# Autodesk Inventor assembly: 64mm_EDF
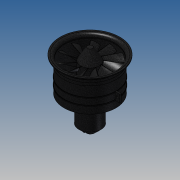
[picture p0: Inventor's stored thumbnail of the model, 180x180]
Saved by Autodesk Inventor 2015 (Build 190159000, 159)
## iProperties
Created: 2018-12-11
Part Number: 64mm_EDF
Document SubType Name: Assembly
Designer: USER
Author: USER
## Documents named in this file (5)
- D:\1102103229\碩士班\論文\Inventor\Drone_twincopterEDF_總組立\64mmEDF_總組立圖4.5\64mm_EDF_3D\64mm_EDF.iam
- D:\1102103229\碩士班\論文\Inventor\Drone_twincopterEDF_總組立\64mmEDF_總組立圖4.5\64mm_EDF_3D\64mm_motor.ipt
- D:\1102103229\碩士班\論文\Inventor\Drone_twincopterEDF_總組立\64mmEDF_總組立圖4.5\64mm_EDF_3D\64mm風扇本體.ipt
- D:\1102103229\碩士班\論文\Inventor\Drone_twincopterEDF_總組立\64mmEDF_總組立圖4.5\64mm_EDF_3D\64mm扇葉.ipt
- D:\1102103229\碩士班\論文\Inventor\Drone_twincopterEDF_總組立\64mmEDF_總組立圖4.5\64mm_EDF_3D\64mm導風口.ipt
## Components (4 placed, 4 different names)
1. 64mm_motor:1 — 貼合:2, 貼合:3, 旋轉:1
2. 64mm風扇本體:1 — 貼合:1, 貼合:2, 貼合:3, 貼合:4, 貼合:5, 齊平:1
3. 64mm扇葉:1 — 貼合:1, 齊平:1, 旋轉:1
4. 64mm導風口:1 — 貼合:4, 貼合:5
## Relationships (7: Mate 5, Flush 1, RelateRotation 1)
- 貼合:1 [Mate]: 64mm風扇本體:1 ↔ 64mm扇葉:1
- 貼合:2 [Mate]: 64mm_motor:1 ↔ 64mm風扇本體:1
- 貼合:3 [Mate]: 64mm_motor:1 ↔ 64mm風扇本體:1
- 貼合:4 [Mate]: 64mm風扇本體:1 ↔ 64mm導風口:1
- 貼合:5 [Mate]: 64mm風扇本體:1 ↔ 64mm導風口:1
- 齊平:1 [Flush] (-13 mm): 64mm風扇本體:1 ↔ 64mm扇葉:1
- 旋轉:1 [RelateRotation] (1 ul): 64mm_motor:1 ↔ 64mm扇葉:1
